# Autodesk Inventor assembly: Assembly2
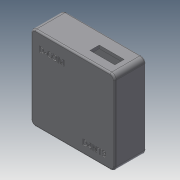
[picture p0: Inventor's stored thumbnail of the model, 180x180]
Saved by Autodesk Inventor 2017 (Build 210142000, 142)
## iProperties
Created: 2020-06-12
Part Number: Assembly2
Document SubType Name: Assembly
Designer: c
Author: c
## Documents named in this file (3)
- C:\Users\c\Desktop\dcom\Assembly2.iam
- C:\Users\c\Desktop\dcom\base.ipt
- C:\Users\c\Desktop\dcom\tapa1.iam
## Components (2 placed, 2 different names)
1. base:1 — Angle:1, Angle:2
2. tapa1:1 [sub-assembly] — Angle:1, Angle:2
## Relationships (2: Angle 2)
- Angle:1 (0 deg): base:1 ↔ tapa1:1
- Angle:2 (0 deg): base:1 ↔ tapa1:1
